# Autodesk Inventor assembly: RT_FRM_A_002
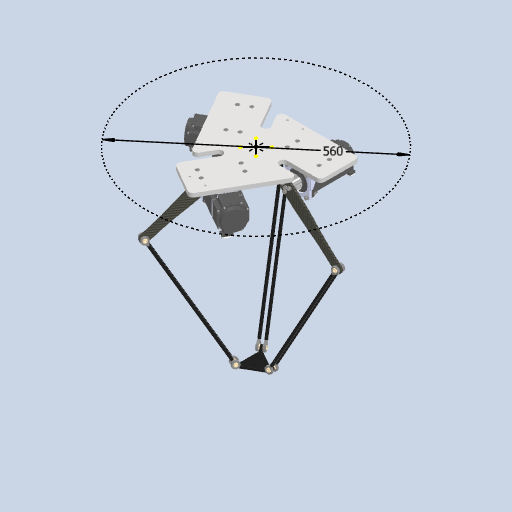
[picture p0: Inventor's stored thumbnail of the model, 512x512]
Saved by Autodesk Inventor 2025.3 (Build 293356000, 356)
## iProperties
Created: 2026-05-11
Part Number: RT_FRM_A_002
Document SubType Name: Assembly
Designer: louis
Mass: 9176.21 g
Surface Area: 8073.41 cm^2
Volume: 2320.58 cm^3
Density: 3.95427 g/cm^3
Author: louis
## Documents named in this file (7)
- C:\Users\louis\OneDrive\Desktop\R_Trident\02_CAD\04_Subassemblies\RT_FRM_A_002_Dynamics.iam
- C:\Users\louis\OneDrive\Desktop\R_Trident\02_CAD\03_Parts_Custom\RT_FRM_MC_004_TopPlate.ipt
- C:\Users\louis\OneDrive\Desktop\R_Trident\02_CAD\04_Subassemblies\RT_ARM_A_001.iam
- C:\Users\louis\OneDrive\Desktop\R_Trident\02_CAD\04_Subassemblies\RT_ARM_A_003.iam
- C:\Users\louis\OneDrive\Desktop\R_Trident\02_CAD\03_Parts_Custom\RT_ARM_MC_007_EndEffector.ipt
- C:\Users\louis\OneDrive\Documents\Inventor\Content Center Files\R2025\en-US\ISO 4762(2)\ISO 4762 - M5 x 20ISO.ipt
- C:\Users\louis\OneDrive\Documents\Inventor\Content Center Files\R2025\en-US\ISO 4032(2)\ISO 4032 - M5 - ISO.ipt
## Components (35 placed, 6 different names)
1. RT_FRM_MC_004_TopPlate:1 — Mate:1, Flush:3, Mate:3, Mate:4, Mate:5, Mate:6, Mate:7, Mate:8, Mate:9, Insert:1, Insert:2, Insert:3, Insert:4, Insert:5, Insert:6, Insert:7, Insert:8, Insert:9, Insert:10, Insert:11, Insert:12, Mate:100
2. RT_ARM_A_001:1 [sub-assembly] — Mate:4, Mate:5, Mate:14, Mate:77, Mate:79, Mate:97, Mate:99, Rotational:9, Rotational:12
3. RT_ARM_A_001:2 [sub-assembly] — Mate:6, Mate:7, Mate:15, Mate:81, Mate:83, Mate:85, Mate:87, Rotational:1, Rotational:3
4. RT_ARM_A_001:3 [sub-assembly] — Mate:8, Mate:9, Mate:16, Mate:89, Mate:91, Mate:93, Mate:95, Rotational:5, Rotational:7
5. RT_ARM_A_003:6 [sub-assembly] — Rotational:11, Rotational:12
6. RT_ARM_A_003:5 [sub-assembly] — Rotational:9, Rotational:10
7. RT_ARM_A_003:4 [sub-assembly] — Rotational:7, Rotational:8
8. RT_ARM_A_003:3 [sub-assembly] — Rotational:5, Rotational:6
9. RT_ARM_A_003:2 [sub-assembly] — Rotational:3, Rotational:4
10. RT_ARM_A_003:1 [sub-assembly] — Rotational:1, Rotational:2
11. RT_ARM_MC_007_EndEffector:1 — Rotational:2, Rotational:4, Rotational:6, Rotational:8, Rotational:10, Rotational:11, Mate:100
12. ISO 4762 M5 x 20:1 — Insert:1, Mate:76
13. ISO 4762 M5 x 20:2 — Insert:2, Mate:82
14. ISO 4762 M5 x 20:3 — Insert:3, Mate:84
15. ISO 4762 M5 x 20:4 — Insert:4, Mate:80
16. ISO 4762 M5 x 20:5 — Insert:5, Mate:86
17. ISO 4762 M5 x 20:6 — Insert:6, Mate:96
18. ISO 4762 M5 x 20:7 — Insert:7, Mate:78
19. ISO 4762 M5 x 20:8 — Insert:8, Mate:98
20. ISO 4762 M5 x 20:9 — Insert:9, Mate:94
21. ISO 4762 M5 x 20:10 — Insert:10, Mate:90
22. ISO 4762 M5 x 20:11 — Insert:11, Mate:92
23. ISO 4762 M5 x 20:12 — Insert:12, Mate:88
24. ISO 4032 M5:1 — Mate:76, Mate:77
25. ISO 4032 M5:2 — Mate:78, Mate:79
26. ISO 4032 M5:3 — Mate:80, Mate:81
27. ISO 4032 M5:4 — Mate:82, Mate:83
28. ISO 4032 M5:5 — Mate:84, Mate:85
29. ISO 4032 M5:6 — Mate:86, Mate:87
30. ISO 4032 M5:7 — Mate:88, Mate:89
31. ISO 4032 M5:8 — Mate:90, Mate:91
32. ISO 4032 M5:9 — Mate:92, Mate:93
33. ISO 4032 M5:10 — Mate:94, Mate:95
34. ISO 4032 M5:11 — Mate:96, Mate:97
35. ISO 4032 M5:12 — Mate:98, Mate:99
## Relationships (62: Mate 36, Insert 12, RevoluteJoint 12, Flush 2)
- Mate:1: RT_FRM_MC_004_TopPlate:1
- Flush:3: RT_FRM_MC_004_TopPlate:1
- Mate:3: RT_FRM_MC_004_TopPlate:1
- Mate:4: RT_FRM_MC_004_TopPlate:1 ↔ RT_ARM_A_001:1
- Mate:5: RT_FRM_MC_004_TopPlate:1 ↔ RT_ARM_A_001:1
- Mate:6: RT_FRM_MC_004_TopPlate:1 ↔ RT_ARM_A_001:2
- Mate:7: RT_FRM_MC_004_TopPlate:1 ↔ RT_ARM_A_001:2
- Mate:8: RT_FRM_MC_004_TopPlate:1 ↔ RT_ARM_A_001:3
- Mate:9: RT_FRM_MC_004_TopPlate:1 ↔ RT_ARM_A_001:3
- Mate:14: RT_ARM_A_001:1
- Mate:15: RT_ARM_A_001:2
- Mate:16: RT_ARM_A_001:3
- Flush:1 (700 mm)
- Insert:1: RT_FRM_MC_004_TopPlate:1 ↔ ISO 4762 M5 x 20:1
- Insert:2: RT_FRM_MC_004_TopPlate:1 ↔ ISO 4762 M5 x 20:2
- Insert:3: RT_FRM_MC_004_TopPlate:1 ↔ ISO 4762 M5 x 20:3
- Insert:4: RT_FRM_MC_004_TopPlate:1 ↔ ISO 4762 M5 x 20:4
- Insert:5: RT_FRM_MC_004_TopPlate:1 ↔ ISO 4762 M5 x 20:5
- Insert:6: RT_FRM_MC_004_TopPlate:1 ↔ ISO 4762 M5 x 20:6
- Insert:7: RT_FRM_MC_004_TopPlate:1 ↔ ISO 4762 M5 x 20:7
- Insert:8: RT_FRM_MC_004_TopPlate:1 ↔ ISO 4762 M5 x 20:8
- Insert:9: RT_FRM_MC_004_TopPlate:1 ↔ ISO 4762 M5 x 20:9
- Insert:10: RT_FRM_MC_004_TopPlate:1 ↔ ISO 4762 M5 x 20:10
- Insert:11: RT_FRM_MC_004_TopPlate:1 ↔ ISO 4762 M5 x 20:11
- Insert:12: RT_FRM_MC_004_TopPlate:1 ↔ ISO 4762 M5 x 20:12
- Mate:76: ISO 4762 M5 x 20:1 ↔ ISO 4032 M5:1
- Mate:77: RT_ARM_A_001:1 ↔ ISO 4032 M5:1
- Mate:78: ISO 4762 M5 x 20:7 ↔ ISO 4032 M5:2
- Mate:79: RT_ARM_A_001:1 ↔ ISO 4032 M5:2
- Mate:80: ISO 4762 M5 x 20:4 ↔ ISO 4032 M5:3
- Mate:81: RT_ARM_A_001:2 ↔ ISO 4032 M5:3
- Mate:82: ISO 4762 M5 x 20:2 ↔ ISO 4032 M5:4
- Mate:83: RT_ARM_A_001:2 ↔ ISO 4032 M5:4
- Mate:84: ISO 4762 M5 x 20:3 ↔ ISO 4032 M5:5
- Mate:85: RT_ARM_A_001:2 ↔ ISO 4032 M5:5
- Mate:86: ISO 4762 M5 x 20:5 ↔ ISO 4032 M5:6
- Mate:87: RT_ARM_A_001:2 ↔ ISO 4032 M5:6
- Mate:88: ISO 4762 M5 x 20:12 ↔ ISO 4032 M5:7
- Mate:89: RT_ARM_A_001:3 ↔ ISO 4032 M5:7
- Mate:90: ISO 4762 M5 x 20:10 ↔ ISO 4032 M5:8
- Mate:91: RT_ARM_A_001:3 ↔ ISO 4032 M5:8
- Mate:92: ISO 4762 M5 x 20:11 ↔ ISO 4032 M5:9
- Mate:93: RT_ARM_A_001:3 ↔ ISO 4032 M5:9
- Mate:94: ISO 4762 M5 x 20:9 ↔ ISO 4032 M5:10
- Mate:95: RT_ARM_A_001:3 ↔ ISO 4032 M5:10
- Mate:96: ISO 4762 M5 x 20:6 ↔ ISO 4032 M5:11
- Mate:97: RT_ARM_A_001:1 ↔ ISO 4032 M5:11
- Mate:98: ISO 4762 M5 x 20:8 ↔ ISO 4032 M5:12
- Mate:99: RT_ARM_A_001:1 ↔ ISO 4032 M5:12
- Rotational:1 [RevoluteJoint]: RT_ARM_A_001:2 ↔ RT_ARM_A_003:1
- Rotational:2 [RevoluteJoint]: RT_ARM_A_003:1 ↔ RT_ARM_MC_007_EndEffector:1
- Rotational:3 [RevoluteJoint]: RT_ARM_A_001:2 ↔ RT_ARM_A_003:2
- Rotational:4 [RevoluteJoint]: RT_ARM_A_003:2 ↔ RT_ARM_MC_007_EndEffector:1
- Rotational:5 [RevoluteJoint]: RT_ARM_A_001:3 ↔ RT_ARM_A_003:3
- Rotational:6 [RevoluteJoint]: RT_ARM_A_003:3 ↔ RT_ARM_MC_007_EndEffector:1
- Rotational:7 [RevoluteJoint]: RT_ARM_A_001:3 ↔ RT_ARM_A_003:4
- Rotational:8 [RevoluteJoint]: RT_ARM_A_003:4 ↔ RT_ARM_MC_007_EndEffector:1
- Rotational:9 [RevoluteJoint]: RT_ARM_A_001:1 ↔ RT_ARM_A_003:5
- Rotational:10 [RevoluteJoint]: RT_ARM_A_003:5 ↔ RT_ARM_MC_007_EndEffector:1
- Rotational:11 [RevoluteJoint]: RT_ARM_A_003:6 ↔ RT_ARM_MC_007_EndEffector:1
- Rotational:12 [RevoluteJoint]: RT_ARM_A_001:1 ↔ RT_ARM_A_003:6
- Mate:100 (540 mm): RT_FRM_MC_004_TopPlate:1 ↔ RT_ARM_MC_007_EndEffector:1
